# Autodesk Inventor assembly: Shooter Assembly v2
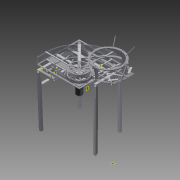
[picture p0: Inventor's stored thumbnail of the model, 180x180]
Saved by Autodesk Inventor 2013 (Build 170138000, 138)
## iProperties
Created: 2013-01-15
Part Number: Shooter Assembly v2
Document SubType Name: Assembly
Designer: actoennies
Mass: 8056.1 g
Surface Area: 23883.9 cm^2
Volume: 3889.96 cm^3
Density: 2.071 g/cm^3
Author: actoennies
## Documents named in this file (34)
- C:\Users\Arpan\Documents\GitHub\frc2013CAD\Launcher\Shooter\Shooter Assembly v2.iam
- C:\Users\Arpan\Documents\GitHub\frc2013CAD\Launcher\Shooter\Bearing Mount v1.ipt
- C:\Users\Arpan\Documents\GitHub\frc2013CAD\Launcher\Shooter\Outer Rail v1.ipt
- C:\Users\Arpan\Documents\GitHub\frc2013CAD\Launcher\Shooter\Runner Rails v2.ipt
- C:\Users\Arpan\Documents\GitHub\frc2013CAD\Launcher\Shooter\Bearing.ipt
- C:\Users\Arpan\Documents\GitHub\frc2013CAD\Launcher\Shooter\Flywheel Assembly.iam
- C:\Users\Arpan\Documents\GitHub\frc2013CAD\Launcher\Shooter\Shooter Mounter.ipt
- C:\Users\Arpan\Documents\GitHub\frc2013CAD\Launcher\Shooter\Bearing Mount 2 v1.ipt
- C:\Users\Arpan\Documents\GitHub\frc2013CAD\Launcher\Shooter\Shorter Shaft.ipt
- C:\Users\Arpan\Documents\GitHub\frc2013CAD\Launcher\Shooter\Spacer Rube.ipt
- C:\Users\Arpan\Documents\GitHub\frc2013CAD\Launcher\Shooter\Edge Mount.ipt
- C:\Users\Arpan\Documents\GitHub\frc2013CAD\Launcher\Shooter\Square Tube.ipt
- C:\Users\Arpan\Documents\GitHub\frc2013CAD\Launcher\Shooter\Flange Bearing Mount Tower.ipt
- C:\Users\Arpan\Documents\GitHub\frc2013CAD\Launcher\Shooter\Flange Bearing Mount Tower Mirror.ipt
- C:\Users\Arpan\Documents\GitHub\frc2013CAD\Launcher\Shooter\Bearing Mount Top.ipt
- C:\Users\Arpan\Documents\GitHub\frc2013CAD\Launcher\Shooter\Square Motor Mount.ipt
- C:\Users\Arpan\Documents\GitHub\frc2013CAD\Launcher\Hopper\HopperAssembly42inch_v5.iam
- C:\Users\Arpan\Documents\GitHub\frc2013CAD\Launcher\Shooter\Shooter Assembly v2\Design Accelerator\Spur Gears1.iam
- C:\Users\Arpan\Documents\GitHub\frc2013CAD\Launcher\Parts\Imported Components\Snow Blower Motor\Snow Blower Motor.iam
- C:\Users\Arpan\Documents\GitHub\frc2013CAD\Launcher\Shooter\Snowblower Motor Mount.ipt
- C:\Users\Arpan\Documents\GitHub\frc2013CAD\Launcher\Shooter\Edge Mount Interference.ipt
- C:\Users\Arpan\Documents\GitHub\frc2013CAD\Launcher\Shooter\8mm shaft.ipt
- C:\Users\Arpan\Documents\GitHub\frc2013CAD\Launcher\Shooter\CIM Bearing.ipt
- C:\Users\Arpan\Documents\GitHub\frc2013CAD\Launcher\Parts\8 Plaction Wheel.iam
- C:\Users\Arpan\Documents\GitHub\frc2013CAD\Launcher\Shooter\Square Tube 2.ipt
- C:\Users\Arpan\Documents\GitHub\frc2013CAD\Launcher\Parts\CIM Motor\Motors_FR801-001.iam
- C:\Users\Arpan\Documents\GitHub\frc2013CAD\Launcher\Shooter\Cim Mount.ipt
- C:\Users\Arpan\Documents\GitHub\frc2013CAD\Launcher\Shooter\Hub v1.ipt
- C:\Users\Arpan\Documents\GitHub\frc2013CAD\Launcher\Shooter\Camera Traffic Light Mount.ipt
- C:\Users\Arpan\Documents\GitHub\frc2013CAD\Launcher\Shooter\Camera Gusset Plat.ipt
- \\NNHSSRV2.hs.sd203.org\ACToennies$\Inventor\Camera.ipt
- C:\Users\Arpan\Documents\GitHub\frc2013CAD\Launcher\Shooter\Square Tube 3.ipt
- C:\Users\Arpan\Documents\GitHub\frc2013CAD\Launcher\Shooter\Square Tube 4.ipt
- C:\Users\Arpan\Documents\GitHub\frc2013CAD\Launcher\Shooter\edge mount shortened.ipt
## Components (40 placed, 33 different names)
1. Bearing Mount v1:1 — Insert:12, Insert:13, Insert:14, Insert:15, Insert:26, Insert:27, Mate:62, Mate:63
2. Outer Rail v1:1 — Insert:12, Insert:13, Insert:47, Insert:48, Flush:21, Mate:87
3. Runner Rails v2:1 — Insert:14, Insert:15, Mate:42
4. Flywheel Assembly:1 [sub-assembly] — Mate:61, Flush:30, Mate:68, Flush:31
5. Shooter Mounter:1 — Insert:26, Insert:27, Insert:34, Flush:11, Insert:35, Insert:36, Insert:37, Insert:38, Flush:19, Mate:45, Flush:24, Flush:40
6. Spacer Rube:1 — Insert:34, Flush:11
7. Bearing Mount 2 v1:1 — Insert:37, Insert:38, Insert:40
8. Bearing Mount 2 v1:2 — Insert:35, Insert:36, Insert:39
9. Bearing:3 — Insert:40, Flush:13, Mate:14, Mate:15
10. Bearing:4 — Insert:39, Flush:12, Mate:12, Mate:13, Mate:36, Mate:44
11. Shorter Shaft:1 — Flush:12, Mate:12, Mate:13, Mate:37
12. Shorter Shaft:2 — Flush:13, Mate:14, Mate:15, Mate:38
13. Edge Mount:2 — Flush:34, Mate:104, Flush:48, Mate:105, Mate:106
14. Square Tube:2 — Insert:41, Insert:42, Flush:19, Flush:23, Flush:26, Mate:50, Mate:52, Flush:27, Mate:81, Flush:32, Mate:93, Flush:41, Flush:42, Mate:125, Mate:126
15. Flange Bearing Mount Tower:1 — Insert:41, Insert:42, Insert:43
16. Bearing:5 — Insert:43, Mate:36, Mate:37
17. Flange Bearing Mount Tower Mirror:1 — Insert:46, Flush:29
18. Bearing:6 — Insert:46, Mate:38
19. Bearing Mount Top:1 — Insert:47, Insert:48, Mate:65, Mate:66, Mate:68
20. Square Motor Mount:1 — Flush:23, Mate:47, Mate:51, Flush:27, Mate:77
21. HopperAssembly42inch_v5:1 [sub-assembly] — Mate:42, Flush:21, Mate:87
22. Spur Gears:1 [sub-assembly] — Mate:44, Mate:45, Flush:24, Flush:25, Mate:46, Angle:2
23. Snow Blower Motor:1 [sub-assembly] — Flush:25, Mate:46, Angle:2, Insert:50, Insert:51
24. Snowblower Motor Mount:1 — Insert:50, Insert:51, Mate:47, Mate:51, Mate:52
25. Edge Mount Interference:1 — Flush:26, Mate:50, Mate:77, Mate:95, Flush:44, Flush:45, Flush:46
26. 8mm shaft:1 — Mate:61, Flush:30, Mate:67, Flush:31, Mate:82, Mate:83, Mate:84, Mate:86
27. CIM Bearing:1 — Mate:65, Mate:66, Mate:67
28. CIM Bearing:2 — Mate:62, Mate:63, Insert:56
29. 8 Plaction Wheel:1 [sub-assembly] — Mate:88, Mate:89, Mate:90, Mate:91, Mate:92
30. Square Tube 2:1 — Mate:81, Flush:32, Flush:34, Mate:106, Mate:107, Mate:124, Flush:49, Mate:126
31. Motors_FR801-001:1 [sub-assembly] — Mate:82, Mate:83, Mate:84, Insert:58
32. Cim Mount:1 — Insert:58, Flush:40
33. Hub v1:1 — Mate:88, Mate:89, Mate:90, Flush:38
34. Hub v1:2 — Mate:91, Flush:38, Mate:92, Insert:56
35. Camera Traffic Light Mount:1 — Mate:93, Flush:41, Flush:42, Mate:94, Flush:43, Mate:101, Mate:102, Mate:103
36. Camera Gusset Plat:1 — Mate:94, Mate:95, Flush:43
37. Camera:1 — Mate:101, Mate:102, Mate:103
38. Square Tube 3:1 — Mate:104, Flush:48, Mate:105, Mate:107, Mate:117, Mate:121, Mate:123
39. Square Tube 4:1 — Mate:117, Mate:121, Mate:122
40. edge mount shortened:1 — Mate:124, Mate:125, Flush:49
## Relationships (100: Mate 51, Flush 25, Insert 23, Angle 1)
- Insert:12: Bearing Mount v1:1 ↔ Outer Rail v1:1
- Insert:13: Bearing Mount v1:1 ↔ Outer Rail v1:1
- Insert:14: Bearing Mount v1:1 ↔ Runner Rails v2:1
- Insert:15: Bearing Mount v1:1 ↔ Runner Rails v2:1
- Insert:26: Bearing Mount v1:1 ↔ Shooter Mounter:1
- Insert:27: Bearing Mount v1:1 ↔ Shooter Mounter:1
- Insert:34: Shooter Mounter:1 ↔ Spacer Rube:1
- Flush:11: Shooter Mounter:1 ↔ Spacer Rube:1
- Insert:35: Shooter Mounter:1 ↔ Bearing Mount 2 v1:2
- Insert:36: Shooter Mounter:1 ↔ Bearing Mount 2 v1:2
- Insert:37: Shooter Mounter:1 ↔ Bearing Mount 2 v1:1
- Insert:38: Shooter Mounter:1 ↔ Bearing Mount 2 v1:1
- Insert:39: Bearing Mount 2 v1:2 ↔ Bearing:4
- Insert:40: Bearing Mount 2 v1:1 ↔ Bearing:3
- Flush:12 (-25.4 mm): Bearing:4 ↔ Shorter Shaft:1
- Mate:12: Bearing:4 ↔ Shorter Shaft:1
- Mate:13: Bearing:4 ↔ Shorter Shaft:1
- Flush:13 (-25.4 mm): Bearing:3 ↔ Shorter Shaft:2
- Mate:14: Bearing:3 ↔ Shorter Shaft:2
- Mate:15: Bearing:3 ↔ Shorter Shaft:2
- Insert:41: Square Tube:2 ↔ Flange Bearing Mount Tower:1
- Insert:42: Square Tube:2 ↔ Flange Bearing Mount Tower:1
- Insert:43: Flange Bearing Mount Tower:1 ↔ Bearing:5
- Flush:19: Shooter Mounter:1 ↔ Square Tube:2
- Mate:36: Bearing:4 ↔ Bearing:5
- Mate:37: Shorter Shaft:1 ↔ Bearing:5
- Insert:46: Flange Bearing Mount Tower Mirror:1 ↔ Bearing:6
- Mate:38: Shorter Shaft:2 ↔ Bearing:6
- Insert:47: Outer Rail v1:1 ↔ Bearing Mount Top:1
- Insert:48: Outer Rail v1:1 ↔ Bearing Mount Top:1
- Mate:42: Runner Rails v2:1 ↔ HopperAssembly42inch_v5:1
- Flush:21: Outer Rail v1:1 ↔ HopperAssembly42inch_v5:1
- Flush:23 (152.4 mm): Square Tube:2 ↔ Square Motor Mount:1
- Mate:44: Bearing:4 ↔ Spur Gears:1
- Mate:45 (25.4 mm): Shooter Mounter:1 ↔ Spur Gears:1
- Flush:24: Shooter Mounter:1 ↔ Spur Gears:1
- Flush:25 (-3.175 mm): Spur Gears:1 ↔ Snow Blower Motor:1
- Mate:46: Spur Gears:1 ↔ Snow Blower Motor:1
- Angle:2 (0 deg): Spur Gears:1 ↔ Snow Blower Motor:1
- Insert:50: Snow Blower Motor:1 ↔ Snowblower Motor Mount:1
- Insert:51: Snow Blower Motor:1 ↔ Snowblower Motor Mount:1
- Mate:47: Square Motor Mount:1 ↔ Snowblower Motor Mount:1
- Flush:26: Square Tube:2 ↔ Edge Mount Interference:1
- Mate:50: Square Tube:2 ↔ Edge Mount Interference:1
- Mate:51: Square Motor Mount:1 ↔ Snowblower Motor Mount:1
- Mate:52: Square Tube:2 ↔ Snowblower Motor Mount:1
- Flush:27: Square Tube:2 ↔ Square Motor Mount:1
- Flush:29 (203.2 mm): Flange Bearing Mount Tower Mirror:1
- Mate:61: Flywheel Assembly:1 ↔ 8mm shaft:1
- Flush:30 (12.7 mm): Flywheel Assembly:1 ↔ 8mm shaft:1
- Mate:62: Bearing Mount v1:1 ↔ CIM Bearing:2
- Mate:63: Bearing Mount v1:1 ↔ CIM Bearing:2
- Mate:65: Bearing Mount Top:1 ↔ CIM Bearing:1
- Mate:66: Bearing Mount Top:1 ↔ CIM Bearing:1
- Mate:67: 8mm shaft:1 ↔ CIM Bearing:1
- Mate:68 (6.35 mm): Flywheel Assembly:1 ↔ Bearing Mount Top:1
- Flush:31: Flywheel Assembly:1 ↔ 8mm shaft:1
- Mate:77: Square Motor Mount:1 ↔ Edge Mount Interference:1
- Mate:81: Square Tube:2 ↔ Square Tube 2:1
- Flush:32: Square Tube:2 ↔ Square Tube 2:1
- Flush:34: Edge Mount:2 ↔ Square Tube 2:1
- Mate:82: 8mm shaft:1 ↔ Motors_FR801-001:1
- Mate:83: 8mm shaft:1 ↔ Motors_FR801-001:1
- Mate:84: 8mm shaft:1 ↔ Motors_FR801-001:1
- Mate:86: 8mm shaft:1
- Mate:87 (25.4 mm): Outer Rail v1:1 ↔ HopperAssembly42inch_v5:1
- Mate:88: 8 Plaction Wheel:1 ↔ Hub v1:1
- Mate:89: 8 Plaction Wheel:1 ↔ Hub v1:1
- Mate:90: 8 Plaction Wheel:1 ↔ Hub v1:1
- Mate:91: 8 Plaction Wheel:1 ↔ Hub v1:2
- Flush:38: Hub v1:1 ↔ Hub v1:2
- Mate:92: 8 Plaction Wheel:1 ↔ Hub v1:2
- Insert:56 (3.175 mm): CIM Bearing:2 ↔ Hub v1:2
- Insert:58: Motors_FR801-001:1 ↔ Cim Mount:1
- Flush:40: Shooter Mounter:1 ↔ Cim Mount:1
- Mate:93: Square Tube:2 ↔ Camera Traffic Light Mount:1
- Flush:41: Square Tube:2 ↔ Camera Traffic Light Mount:1
- Flush:42: Square Tube:2 ↔ Camera Traffic Light Mount:1
- Mate:94: Camera Traffic Light Mount:1 ↔ Camera Gusset Plat:1
- Mate:95: Edge Mount Interference:1 ↔ Camera Gusset Plat:1
- Flush:43 (11.1125 mm): Camera Traffic Light Mount:1 ↔ Camera Gusset Plat:1
- Flush:44 (-203.2 mm): Edge Mount Interference:1
- Flush:45 (-508 mm): Edge Mount Interference:1
- Flush:46 (-660.4 mm): Edge Mount Interference:1
- Mate:101: Camera Traffic Light Mount:1 ↔ Camera:1
- Mate:102: Camera Traffic Light Mount:1 ↔ Camera:1
- Mate:103: Camera Traffic Light Mount:1 ↔ Camera:1
- Mate:104: Edge Mount:2 ↔ Square Tube 3:1
- Flush:48: Edge Mount:2 ↔ Square Tube 3:1
- Mate:105: Edge Mount:2 ↔ Square Tube 3:1
- Mate:106: Edge Mount:2 ↔ Square Tube 2:1
- Mate:107: Square Tube 2:1 ↔ Square Tube 3:1
- Mate:117: Square Tube 3:1 ↔ Square Tube 4:1
- Mate:121: Square Tube 3:1 ↔ Square Tube 4:1
- Mate:122: Square Tube 4:1
- Mate:123: Square Tube 3:1
- Mate:124: Square Tube 2:1 ↔ edge mount shortened:1
- Mate:125: Square Tube:2 ↔ edge mount shortened:1
- Flush:49: Square Tube 2:1 ↔ edge mount shortened:1
- Mate:126: Square Tube:2 ↔ Square Tube 2:1
